# Autodesk Inventor assembly: AmpPS
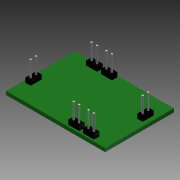
[picture p0: Inventor's stored thumbnail of the model, 180x180]
Saved by Autodesk Inventor 2014 (Build 180170000, 170)
## iProperties
Created: 2015-04-19
Part Number: AmpPS
Document SubType Name: Assembly
Designer: Owner
Author: Owner
## Documents named in this file (3)
- C:\Users\Owner\Documents\APC\FrontEnd\IAM\Common\AmpPS.iam
- C:\Users\Owner\Documents\APC\FrontEnd\IAM\Common\AmpPSBoard.ipt
- C:\Users\Owner\Documents\APC\FrontEnd\IAM\Common\2PinHeader.ipt
## Components (7 placed, 2 different names)
1. AmpPSBoard:1 — Mate:1, Mate:2, Mate:3, Mate:4, Mate:5, Mate:6, Flush:1, Flush:2, Flush:3, Flush:4, Flush:5, Flush:6, Flush:7, Flush:8, Flush:9, Flush:10, Flush:11, Flush:12
2. 2PinHeader:1 — Mate:3, Flush:3, Flush:9
3. 2PinHeader:2 — Mate:2, Flush:2, Flush:8
4. 2PinHeader:3 — Mate:4, Flush:6, Flush:12
5. 2PinHeader:4 — Mate:1, Flush:1, Flush:7
6. 2PinHeader:5 — Mate:5, Flush:4, Flush:11
7. 2PinHeader:6 — Mate:6, Flush:5, Flush:10
## Relationships (18: Flush 12, Mate 6)
- Mate:1: AmpPSBoard:1 ↔ 2PinHeader:4
- Mate:2: AmpPSBoard:1 ↔ 2PinHeader:2
- Mate:3: AmpPSBoard:1 ↔ 2PinHeader:1
- Mate:4: AmpPSBoard:1 ↔ 2PinHeader:3
- Mate:5: AmpPSBoard:1 ↔ 2PinHeader:5
- Mate:6: AmpPSBoard:1 ↔ 2PinHeader:6
- Flush:1 (0.8128 mm): AmpPSBoard:1 ↔ 2PinHeader:4
- Flush:2 (0.8128 mm): AmpPSBoard:1 ↔ 2PinHeader:2
- Flush:3 (1.8288 mm): AmpPSBoard:1 ↔ 2PinHeader:1
- Flush:4 (0.5588 mm): AmpPSBoard:1 ↔ 2PinHeader:5
- Flush:5 (0.5588 mm): AmpPSBoard:1 ↔ 2PinHeader:6
- Flush:6 (1.0668 mm): AmpPSBoard:1 ↔ 2PinHeader:3
- Flush:7 (5.969 mm): AmpPSBoard:1 ↔ 2PinHeader:4
- Flush:8 (12.8016 mm): AmpPSBoard:1 ↔ 2PinHeader:2
- Flush:9 (19.177 mm): AmpPSBoard:1 ↔ 2PinHeader:1
- Flush:10 (25.527 mm): AmpPSBoard:1 ↔ 2PinHeader:6
- Flush:11 (32.3596 mm): AmpPSBoard:1 ↔ 2PinHeader:5
- Flush:12 (7.7216 mm): AmpPSBoard:1 ↔ 2PinHeader:3
